(part 1 of 2)
# Autodesk Inventor assembly: NanoPower P31u-9
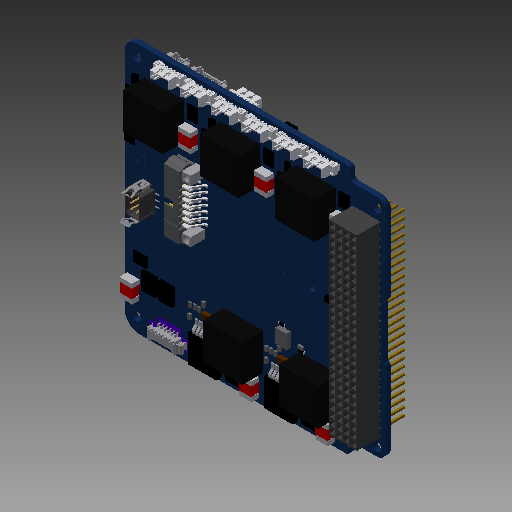
[picture p0: Inventor's stored thumbnail of the model, 512x512]
Saved by Autodesk Inventor 2017 (Build 210142000, 142)
## iProperties
Created: 2014-06-10
Part Number: NanoPower P31u-9
Document SubType Name: Assembly
Designer: Cosmonauta
Sending System: Autodesk Inventor 2014
Preprocessor: ST-DEVELOPER v15.2
Title: \\psf\Home\Desktop\NanoPower P31u-9.stp
Author: David
## Documents named in this file (322)
- C:\Users\Cosmonauta\ownCloud\Aurora\Proyectos\SUCHAI_2-3\Subsistemas\MEC\CAD_Cubesat3U\Nanopower_P31U\CAD\NanoPower P31u-9.iam
- C:\Users\Cosmonauta\ownCloud\Aurora\Proyectos\SUCHAI_2-3\Subsistemas\MEC\CAD_Cubesat3U\Nanopower_P31U\CAD\Board.ipt
- C:\Users\Cosmonauta\ownCloud\Aurora\Proyectos\SUCHAI_2-3\Subsistemas\MEC\CAD_Cubesat3U\Nanopower_P31U\CAD\R104.iam
- C:\Users\Cosmonauta\ownCloud\Aurora\Proyectos\SUCHAI_2-3\Subsistemas\MEC\CAD_Cubesat3U\Nanopower_P31U\CAD\R701.iam
- C:\Users\Cosmonauta\ownCloud\Aurora\Proyectos\SUCHAI_2-3\Subsistemas\MEC\CAD_Cubesat3U\Nanopower_P31U\CAD\U700.iam
- C:\Users\Cosmonauta\ownCloud\Aurora\Proyectos\SUCHAI_2-3\Subsistemas\MEC\CAD_Cubesat3U\Nanopower_P31U\CAD\R700.iam
- C:\Users\Cosmonauta\ownCloud\Aurora\Proyectos\SUCHAI_2-3\Subsistemas\MEC\CAD_Cubesat3U\Nanopower_P31U\CAD\C700.iam
- C:\Users\Cosmonauta\ownCloud\Aurora\Proyectos\SUCHAI_2-3\Subsistemas\MEC\CAD_Cubesat3U\Nanopower_P31U\CAD\Q411.iam
- C:\Users\Cosmonauta\ownCloud\Aurora\Proyectos\SUCHAI_2-3\Subsistemas\MEC\CAD_Cubesat3U\Nanopower_P31U\CAD\Q410.iam
- C:\Users\Cosmonauta\ownCloud\Aurora\Proyectos\SUCHAI_2-3\Subsistemas\MEC\CAD_Cubesat3U\Nanopower_P31U\CAD\U605.iam
- C:\Users\Cosmonauta\ownCloud\Aurora\Proyectos\SUCHAI_2-3\Subsistemas\MEC\CAD_Cubesat3U\Nanopower_P31U\CAD\U604.iam
- C:\Users\Cosmonauta\ownCloud\Aurora\Proyectos\SUCHAI_2-3\Subsistemas\MEC\CAD_Cubesat3U\Nanopower_P31U\CAD\U603.iam
- C:\Users\Cosmonauta\ownCloud\Aurora\Proyectos\SUCHAI_2-3\Subsistemas\MEC\CAD_Cubesat3U\Nanopower_P31U\CAD\U602.iam
- C:\Users\Cosmonauta\ownCloud\Aurora\Proyectos\SUCHAI_2-3\Subsistemas\MEC\CAD_Cubesat3U\Nanopower_P31U\CAD\R304.iam
- C:\Users\Cosmonauta\ownCloud\Aurora\Proyectos\SUCHAI_2-3\Subsistemas\MEC\CAD_Cubesat3U\Nanopower_P31U\CAD\R303.iam
- C:\Users\Cosmonauta\ownCloud\Aurora\Proyectos\SUCHAI_2-3\Subsistemas\MEC\CAD_Cubesat3U\Nanopower_P31U\CAD\R7_M506.iam
- C:\Users\Cosmonauta\ownCloud\Aurora\Proyectos\SUCHAI_2-3\Subsistemas\MEC\CAD_Cubesat3U\Nanopower_P31U\CAD\R7_M505.iam
- C:\Users\Cosmonauta\ownCloud\Aurora\Proyectos\SUCHAI_2-3\Subsistemas\MEC\CAD_Cubesat3U\Nanopower_P31U\CAD\R7_M504.iam
- C:\Users\Cosmonauta\ownCloud\Aurora\Proyectos\SUCHAI_2-3\Subsistemas\MEC\CAD_Cubesat3U\Nanopower_P31U\CAD\R7_M503.iam
- C:\Users\Cosmonauta\ownCloud\Aurora\Proyectos\SUCHAI_2-3\Subsistemas\MEC\CAD_Cubesat3U\Nanopower_P31U\CAD\R7_M502.iam
- C:\Users\Cosmonauta\ownCloud\Aurora\Proyectos\SUCHAI_2-3\Subsistemas\MEC\CAD_Cubesat3U\Nanopower_P31U\CAD\R7_M501.iam
- C:\Users\Cosmonauta\ownCloud\Aurora\Proyectos\SUCHAI_2-3\Subsistemas\MEC\CAD_Cubesat3U\Nanopower_P31U\CAD\C4_M506.iam
- C:\Users\Cosmonauta\ownCloud\Aurora\Proyectos\SUCHAI_2-3\Subsistemas\MEC\CAD_Cubesat3U\Nanopower_P31U\CAD\C4_M505.iam
- C:\Users\Cosmonauta\ownCloud\Aurora\Proyectos\SUCHAI_2-3\Subsistemas\MEC\CAD_Cubesat3U\Nanopower_P31U\CAD\C4_M504.iam
- C:\Users\Cosmonauta\ownCloud\Aurora\Proyectos\SUCHAI_2-3\Subsistemas\MEC\CAD_Cubesat3U\Nanopower_P31U\CAD\C4_M503.iam
- C:\Users\Cosmonauta\ownCloud\Aurora\Proyectos\SUCHAI_2-3\Subsistemas\MEC\CAD_Cubesat3U\Nanopower_P31U\CAD\C4_M502.iam
- C:\Users\Cosmonauta\ownCloud\Aurora\Proyectos\SUCHAI_2-3\Subsistemas\MEC\CAD_Cubesat3U\Nanopower_P31U\CAD\C4_M501.iam
- C:\Users\Cosmonauta\ownCloud\Aurora\Proyectos\SUCHAI_2-3\Subsistemas\MEC\CAD_Cubesat3U\Nanopower_P31U\CAD\R6_B3.iam
- C:\Users\Cosmonauta\ownCloud\Aurora\Proyectos\SUCHAI_2-3\Subsistemas\MEC\CAD_Cubesat3U\Nanopower_P31U\CAD\R6_B2.iam
- C:\Users\Cosmonauta\ownCloud\Aurora\Proyectos\SUCHAI_2-3\Subsistemas\MEC\CAD_Cubesat3U\Nanopower_P31U\CAD\R6_B1.iam
- C:\Users\Cosmonauta\ownCloud\Aurora\Proyectos\SUCHAI_2-3\Subsistemas\MEC\CAD_Cubesat3U\Nanopower_P31U\CAD\C6_B3.iam
- C:\Users\Cosmonauta\ownCloud\Aurora\Proyectos\SUCHAI_2-3\Subsistemas\MEC\CAD_Cubesat3U\Nanopower_P31U\CAD\C6_B2.iam
- C:\Users\Cosmonauta\ownCloud\Aurora\Proyectos\SUCHAI_2-3\Subsistemas\MEC\CAD_Cubesat3U\Nanopower_P31U\CAD\C6_B1.iam
- C:\Users\Cosmonauta\ownCloud\Aurora\Proyectos\SUCHAI_2-3\Subsistemas\MEC\CAD_Cubesat3U\Nanopower_P31U\CAD\R103.iam
- C:\Users\Cosmonauta\ownCloud\Aurora\Proyectos\SUCHAI_2-3\Subsistemas\MEC\CAD_Cubesat3U\Nanopower_P31U\CAD\R102.iam
- C:\Users\Cosmonauta\ownCloud\Aurora\Proyectos\SUCHAI_2-3\Subsistemas\MEC\CAD_Cubesat3U\Nanopower_P31U\CAD\C103.iam
- C:\Users\Cosmonauta\ownCloud\Aurora\Proyectos\SUCHAI_2-3\Subsistemas\MEC\CAD_Cubesat3U\Nanopower_P31U\CAD\C102.iam
- C:\Users\Cosmonauta\ownCloud\Aurora\Proyectos\SUCHAI_2-3\Subsistemas\MEC\CAD_Cubesat3U\Nanopower_P31U\CAD\R622.iam
- C:\Users\Cosmonauta\ownCloud\Aurora\Proyectos\SUCHAI_2-3\Subsistemas\MEC\CAD_Cubesat3U\Nanopower_P31U\CAD\R621.iam
- C:\Users\Cosmonauta\ownCloud\Aurora\Proyectos\SUCHAI_2-3\Subsistemas\MEC\CAD_Cubesat3U\Nanopower_P31U\CAD\R620.iam
- C:\Users\Cosmonauta\ownCloud\Aurora\Proyectos\SUCHAI_2-3\Subsistemas\MEC\CAD_Cubesat3U\Nanopower_P31U\CAD\R619.iam
- C:\Users\Cosmonauta\ownCloud\Aurora\Proyectos\SUCHAI_2-3\Subsistemas\MEC\CAD_Cubesat3U\Nanopower_P31U\CAD\R414.iam
- C:\Users\Cosmonauta\ownCloud\Aurora\Proyectos\SUCHAI_2-3\Subsistemas\MEC\CAD_Cubesat3U\Nanopower_P31U\CAD\P601.iam
- C:\Users\Cosmonauta\ownCloud\Aurora\Proyectos\SUCHAI_2-3\Subsistemas\MEC\CAD_Cubesat3U\Nanopower_P31U\CAD\U601.iam
- C:\Users\Cosmonauta\ownCloud\Aurora\Proyectos\SUCHAI_2-3\Subsistemas\MEC\CAD_Cubesat3U\Nanopower_P31U\CAD\P600.iam
- C:\Users\Cosmonauta\ownCloud\Aurora\Proyectos\SUCHAI_2-3\Subsistemas\MEC\CAD_Cubesat3U\Nanopower_P31U\CAD\PBAT.iam
- C:\Users\Cosmonauta\ownCloud\Aurora\Proyectos\SUCHAI_2-3\Subsistemas\MEC\CAD_Cubesat3U\Nanopower_P31U\CAD\C4_B50.iam
- C:\Users\Cosmonauta\ownCloud\Aurora\Proyectos\SUCHAI_2-3\Subsistemas\MEC\CAD_Cubesat3U\Nanopower_P31U\CAD\C2_B50.iam
- C:\Users\Cosmonauta\ownCloud\Aurora\Proyectos\SUCHAI_2-3\Subsistemas\MEC\CAD_Cubesat3U\Nanopower_P31U\CAD\U1_M506.iam
- C:\Users\Cosmonauta\ownCloud\Aurora\Proyectos\SUCHAI_2-3\Subsistemas\MEC\CAD_Cubesat3U\Nanopower_P31U\CAD\U1_M505.iam
- C:\Users\Cosmonauta\ownCloud\Aurora\Proyectos\SUCHAI_2-3\Subsistemas\MEC\CAD_Cubesat3U\Nanopower_P31U\CAD\U1_M504.iam
- C:\Users\Cosmonauta\ownCloud\Aurora\Proyectos\SUCHAI_2-3\Subsistemas\MEC\CAD_Cubesat3U\Nanopower_P31U\CAD\U1_M503.iam
- C:\Users\Cosmonauta\ownCloud\Aurora\Proyectos\SUCHAI_2-3\Subsistemas\MEC\CAD_Cubesat3U\Nanopower_P31U\CAD\U1_M502.iam
- C:\Users\Cosmonauta\ownCloud\Aurora\Proyectos\SUCHAI_2-3\Subsistemas\MEC\CAD_Cubesat3U\Nanopower_P31U\CAD\U1_M501.iam
- C:\Users\Cosmonauta\ownCloud\Aurora\Proyectos\SUCHAI_2-3\Subsistemas\MEC\CAD_Cubesat3U\Nanopower_P31U\CAD\C1_B1.iam
- C:\Users\Cosmonauta\ownCloud\Aurora\Proyectos\SUCHAI_2-3\Subsistemas\MEC\CAD_Cubesat3U\Nanopower_P31U\CAD\C1_B2.iam
- C:\Users\Cosmonauta\ownCloud\Aurora\Proyectos\SUCHAI_2-3\Subsistemas\MEC\CAD_Cubesat3U\Nanopower_P31U\CAD\C1_B3.iam
- C:\Users\Cosmonauta\ownCloud\Aurora\Proyectos\SUCHAI_2-3\Subsistemas\MEC\CAD_Cubesat3U\Nanopower_P31U\CAD\C2_B1.iam
- C:\Users\Cosmonauta\ownCloud\Aurora\Proyectos\SUCHAI_2-3\Subsistemas\MEC\CAD_Cubesat3U\Nanopower_P31U\CAD\C2_B2.iam
- C:\Users\Cosmonauta\ownCloud\Aurora\Proyectos\SUCHAI_2-3\Subsistemas\MEC\CAD_Cubesat3U\Nanopower_P31U\CAD\C2_B3.iam
- C:\Users\Cosmonauta\ownCloud\Aurora\Proyectos\SUCHAI_2-3\Subsistemas\MEC\CAD_Cubesat3U\Nanopower_P31U\CAD\C2_B33.iam
- C:\Users\Cosmonauta\ownCloud\Aurora\Proyectos\SUCHAI_2-3\Subsistemas\MEC\CAD_Cubesat3U\Nanopower_P31U\CAD\C3_B1.iam
- C:\Users\Cosmonauta\ownCloud\Aurora\Proyectos\SUCHAI_2-3\Subsistemas\MEC\CAD_Cubesat3U\Nanopower_P31U\CAD\C3_B2.iam
- C:\Users\Cosmonauta\ownCloud\Aurora\Proyectos\SUCHAI_2-3\Subsistemas\MEC\CAD_Cubesat3U\Nanopower_P31U\CAD\C3_B3.iam
- C:\Users\Cosmonauta\ownCloud\Aurora\Proyectos\SUCHAI_2-3\Subsistemas\MEC\CAD_Cubesat3U\Nanopower_P31U\CAD\C3_B33.iam
- C:\Users\Cosmonauta\ownCloud\Aurora\Proyectos\SUCHAI_2-3\Subsistemas\MEC\CAD_Cubesat3U\Nanopower_P31U\CAD\C3_B50.iam
- C:\Users\Cosmonauta\ownCloud\Aurora\Proyectos\SUCHAI_2-3\Subsistemas\MEC\CAD_Cubesat3U\Nanopower_P31U\CAD\C4_B1.iam
- C:\Users\Cosmonauta\ownCloud\Aurora\Proyectos\SUCHAI_2-3\Subsistemas\MEC\CAD_Cubesat3U\Nanopower_P31U\CAD\C4_B2.iam
- C:\Users\Cosmonauta\ownCloud\Aurora\Proyectos\SUCHAI_2-3\Subsistemas\MEC\CAD_Cubesat3U\Nanopower_P31U\CAD\C4_B3.iam
- C:\Users\Cosmonauta\ownCloud\Aurora\Proyectos\SUCHAI_2-3\Subsistemas\MEC\CAD_Cubesat3U\Nanopower_P31U\CAD\C4_B33.iam
- C:\Users\Cosmonauta\ownCloud\Aurora\Proyectos\SUCHAI_2-3\Subsistemas\MEC\CAD_Cubesat3U\Nanopower_P31U\CAD\C5_B33.iam
- C:\Users\Cosmonauta\ownCloud\Aurora\Proyectos\SUCHAI_2-3\Subsistemas\MEC\CAD_Cubesat3U\Nanopower_P31U\CAD\C5_B50.iam
- C:\Users\Cosmonauta\ownCloud\Aurora\Proyectos\SUCHAI_2-3\Subsistemas\MEC\CAD_Cubesat3U\Nanopower_P31U\CAD\C100.iam
- C:\Users\Cosmonauta\ownCloud\Aurora\Proyectos\SUCHAI_2-3\Subsistemas\MEC\CAD_Cubesat3U\Nanopower_P31U\CAD\C101.iam
- C:\Users\Cosmonauta\ownCloud\Aurora\Proyectos\SUCHAI_2-3\Subsistemas\MEC\CAD_Cubesat3U\Nanopower_P31U\CAD\C200.iam
- C:\Users\Cosmonauta\ownCloud\Aurora\Proyectos\SUCHAI_2-3\Subsistemas\MEC\CAD_Cubesat3U\Nanopower_P31U\CAD\C201.iam
- C:\Users\Cosmonauta\ownCloud\Aurora\Proyectos\SUCHAI_2-3\Subsistemas\MEC\CAD_Cubesat3U\Nanopower_P31U\CAD\C202.iam
- C:\Users\Cosmonauta\ownCloud\Aurora\Proyectos\SUCHAI_2-3\Subsistemas\MEC\CAD_Cubesat3U\Nanopower_P31U\CAD\C400.iam
- C:\Users\Cosmonauta\ownCloud\Aurora\Proyectos\SUCHAI_2-3\Subsistemas\MEC\CAD_Cubesat3U\Nanopower_P31U\CAD\D1_B1.iam
- C:\Users\Cosmonauta\ownCloud\Aurora\Proyectos\SUCHAI_2-3\Subsistemas\MEC\CAD_Cubesat3U\Nanopower_P31U\CAD\D1_B2.iam
- C:\Users\Cosmonauta\ownCloud\Aurora\Proyectos\SUCHAI_2-3\Subsistemas\MEC\CAD_Cubesat3U\Nanopower_P31U\CAD\D1_B3.iam
- C:\Users\Cosmonauta\ownCloud\Aurora\Proyectos\SUCHAI_2-3\Subsistemas\MEC\CAD_Cubesat3U\Nanopower_P31U\CAD\D1_B33.iam
- C:\Users\Cosmonauta\ownCloud\Aurora\Proyectos\SUCHAI_2-3\Subsistemas\MEC\CAD_Cubesat3U\Nanopower_P31U\CAD\D1_B50.iam
- C:\Users\Cosmonauta\ownCloud\Aurora\Proyectos\SUCHAI_2-3\Subsistemas\MEC\CAD_Cubesat3U\Nanopower_P31U\CAD\L1_B1.iam
- C:\Users\Cosmonauta\ownCloud\Aurora\Proyectos\SUCHAI_2-3\Subsistemas\MEC\CAD_Cubesat3U\Nanopower_P31U\CAD\L1_B2.iam
- C:\Users\Cosmonauta\ownCloud\Aurora\Proyectos\SUCHAI_2-3\Subsistemas\MEC\CAD_Cubesat3U\Nanopower_P31U\CAD\L1_B3.iam
- C:\Users\Cosmonauta\ownCloud\Aurora\Proyectos\SUCHAI_2-3\Subsistemas\MEC\CAD_Cubesat3U\Nanopower_P31U\CAD\L1_B33.iam
- C:\Users\Cosmonauta\ownCloud\Aurora\Proyectos\SUCHAI_2-3\Subsistemas\MEC\CAD_Cubesat3U\Nanopower_P31U\CAD\L1_B50.iam
- C:\Users\Cosmonauta\ownCloud\Aurora\Proyectos\SUCHAI_2-3\Subsistemas\MEC\CAD_Cubesat3U\Nanopower_P31U\CAD\P100.iam
- C:\Users\Cosmonauta\ownCloud\Aurora\Proyectos\SUCHAI_2-3\Subsistemas\MEC\CAD_Cubesat3U\Nanopower_P31U\CAD\P101.iam
- C:\Users\Cosmonauta\ownCloud\Aurora\Proyectos\SUCHAI_2-3\Subsistemas\MEC\CAD_Cubesat3U\Nanopower_P31U\CAD\P102.iam
- C:\Users\Cosmonauta\ownCloud\Aurora\Proyectos\SUCHAI_2-3\Subsistemas\MEC\CAD_Cubesat3U\Nanopower_P31U\CAD\P103.iam
- C:\Users\Cosmonauta\ownCloud\Aurora\Proyectos\SUCHAI_2-3\Subsistemas\MEC\CAD_Cubesat3U\Nanopower_P31U\CAD\P104.iam
- C:\Users\Cosmonauta\ownCloud\Aurora\Proyectos\SUCHAI_2-3\Subsistemas\MEC\CAD_Cubesat3U\Nanopower_P31U\CAD\P105.iam
- C:\Users\Cosmonauta\ownCloud\Aurora\Proyectos\SUCHAI_2-3\Subsistemas\MEC\CAD_Cubesat3U\Nanopower_P31U\CAD\P400.iam
- C:\Users\Cosmonauta\ownCloud\Aurora\Proyectos\SUCHAI_2-3\Subsistemas\MEC\CAD_Cubesat3U\Nanopower_P31U\CAD\Q1_B1.iam
- C:\Users\Cosmonauta\ownCloud\Aurora\Proyectos\SUCHAI_2-3\Subsistemas\MEC\CAD_Cubesat3U\Nanopower_P31U\CAD\Q1_B2.iam
- C:\Users\Cosmonauta\ownCloud\Aurora\Proyectos\SUCHAI_2-3\Subsistemas\MEC\CAD_Cubesat3U\Nanopower_P31U\CAD\Q1_B3.iam
- C:\Users\Cosmonauta\ownCloud\Aurora\Proyectos\SUCHAI_2-3\Subsistemas\MEC\CAD_Cubesat3U\Nanopower_P31U\CAD\Q2_B1.iam
- C:\Users\Cosmonauta\ownCloud\Aurora\Proyectos\SUCHAI_2-3\Subsistemas\MEC\CAD_Cubesat3U\Nanopower_P31U\CAD\Q2_B2.iam
- C:\Users\Cosmonauta\ownCloud\Aurora\Proyectos\SUCHAI_2-3\Subsistemas\MEC\CAD_Cubesat3U\Nanopower_P31U\CAD\Q2_B3.iam
- C:\Users\Cosmonauta\ownCloud\Aurora\Proyectos\SUCHAI_2-3\Subsistemas\MEC\CAD_Cubesat3U\Nanopower_P31U\CAD\Q200.iam
- C:\Users\Cosmonauta\ownCloud\Aurora\Proyectos\SUCHAI_2-3\Subsistemas\MEC\CAD_Cubesat3U\Nanopower_P31U\CAD\Q201.iam
- C:\Users\Cosmonauta\ownCloud\Aurora\Proyectos\SUCHAI_2-3\Subsistemas\MEC\CAD_Cubesat3U\Nanopower_P31U\CAD\Q400.iam
- C:\Users\Cosmonauta\ownCloud\Aurora\Proyectos\SUCHAI_2-3\Subsistemas\MEC\CAD_Cubesat3U\Nanopower_P31U\CAD\Q401.iam
- C:\Users\Cosmonauta\ownCloud\Aurora\Proyectos\SUCHAI_2-3\Subsistemas\MEC\CAD_Cubesat3U\Nanopower_P31U\CAD\Q402.iam
- C:\Users\Cosmonauta\ownCloud\Aurora\Proyectos\SUCHAI_2-3\Subsistemas\MEC\CAD_Cubesat3U\Nanopower_P31U\CAD\Q404.iam
- C:\Users\Cosmonauta\ownCloud\Aurora\Proyectos\SUCHAI_2-3\Subsistemas\MEC\CAD_Cubesat3U\Nanopower_P31U\CAD\R1_B1.iam
- C:\Users\Cosmonauta\ownCloud\Aurora\Proyectos\SUCHAI_2-3\Subsistemas\MEC\CAD_Cubesat3U\Nanopower_P31U\CAD\R1_B2.iam
- C:\Users\Cosmonauta\ownCloud\Aurora\Proyectos\SUCHAI_2-3\Subsistemas\MEC\CAD_Cubesat3U\Nanopower_P31U\CAD\R1_B3.iam
- C:\Users\Cosmonauta\ownCloud\Aurora\Proyectos\SUCHAI_2-3\Subsistemas\MEC\CAD_Cubesat3U\Nanopower_P31U\CAD\R1_B33.iam
- C:\Users\Cosmonauta\ownCloud\Aurora\Proyectos\SUCHAI_2-3\Subsistemas\MEC\CAD_Cubesat3U\Nanopower_P31U\CAD\R1_B50.iam
- C:\Users\Cosmonauta\ownCloud\Aurora\Proyectos\SUCHAI_2-3\Subsistemas\MEC\CAD_Cubesat3U\Nanopower_P31U\CAD\R2_B1.iam
- C:\Users\Cosmonauta\ownCloud\Aurora\Proyectos\SUCHAI_2-3\Subsistemas\MEC\CAD_Cubesat3U\Nanopower_P31U\CAD\R2_B2.iam
- C:\Users\Cosmonauta\ownCloud\Aurora\Proyectos\SUCHAI_2-3\Subsistemas\MEC\CAD_Cubesat3U\Nanopower_P31U\CAD\R2_B3.iam
- C:\Users\Cosmonauta\ownCloud\Aurora\Proyectos\SUCHAI_2-3\Subsistemas\MEC\CAD_Cubesat3U\Nanopower_P31U\CAD\R2_B33.iam
- C:\Users\Cosmonauta\ownCloud\Aurora\Proyectos\SUCHAI_2-3\Subsistemas\MEC\CAD_Cubesat3U\Nanopower_P31U\CAD\R2_B50.iam
- C:\Users\Cosmonauta\ownCloud\Aurora\Proyectos\SUCHAI_2-3\Subsistemas\MEC\CAD_Cubesat3U\Nanopower_P31U\CAD\R3_B1.iam
- C:\Users\Cosmonauta\ownCloud\Aurora\Proyectos\SUCHAI_2-3\Subsistemas\MEC\CAD_Cubesat3U\Nanopower_P31U\CAD\R3_B2.iam
- C:\Users\Cosmonauta\ownCloud\Aurora\Proyectos\SUCHAI_2-3\Subsistemas\MEC\CAD_Cubesat3U\Nanopower_P31U\CAD\R3_B3.iam
- C:\Users\Cosmonauta\ownCloud\Aurora\Proyectos\SUCHAI_2-3\Subsistemas\MEC\CAD_Cubesat3U\Nanopower_P31U\CAD\R3_B33.iam
- C:\Users\Cosmonauta\ownCloud\Aurora\Proyectos\SUCHAI_2-3\Subsistemas\MEC\CAD_Cubesat3U\Nanopower_P31U\CAD\R3_B50.iam
- C:\Users\Cosmonauta\ownCloud\Aurora\Proyectos\SUCHAI_2-3\Subsistemas\MEC\CAD_Cubesat3U\Nanopower_P31U\CAD\R4_B1.iam
- C:\Users\Cosmonauta\ownCloud\Aurora\Proyectos\SUCHAI_2-3\Subsistemas\MEC\CAD_Cubesat3U\Nanopower_P31U\CAD\R4_B2.iam
- C:\Users\Cosmonauta\ownCloud\Aurora\Proyectos\SUCHAI_2-3\Subsistemas\MEC\CAD_Cubesat3U\Nanopower_P31U\CAD\R4_B3.iam
- C:\Users\Cosmonauta\ownCloud\Aurora\Proyectos\SUCHAI_2-3\Subsistemas\MEC\CAD_Cubesat3U\Nanopower_P31U\CAD\R5_B1.iam
- C:\Users\Cosmonauta\ownCloud\Aurora\Proyectos\SUCHAI_2-3\Subsistemas\MEC\CAD_Cubesat3U\Nanopower_P31U\CAD\R5_B2.iam
- C:\Users\Cosmonauta\ownCloud\Aurora\Proyectos\SUCHAI_2-3\Subsistemas\MEC\CAD_Cubesat3U\Nanopower_P31U\CAD\R5_B3.iam
- C:\Users\Cosmonauta\ownCloud\Aurora\Proyectos\SUCHAI_2-3\Subsistemas\MEC\CAD_Cubesat3U\Nanopower_P31U\CAD\R100.iam
- C:\Users\Cosmonauta\ownCloud\Aurora\Proyectos\SUCHAI_2-3\Subsistemas\MEC\CAD_Cubesat3U\Nanopower_P31U\CAD\R101.iam
- C:\Users\Cosmonauta\ownCloud\Aurora\Proyectos\SUCHAI_2-3\Subsistemas\MEC\CAD_Cubesat3U\Nanopower_P31U\CAD\R107_B1.iam
- C:\Users\Cosmonauta\ownCloud\Aurora\Proyectos\SUCHAI_2-3\Subsistemas\MEC\CAD_Cubesat3U\Nanopower_P31U\CAD\R107_B2.iam
- C:\Users\Cosmonauta\ownCloud\Aurora\Proyectos\SUCHAI_2-3\Subsistemas\MEC\CAD_Cubesat3U\Nanopower_P31U\CAD\R107_B3.iam
- C:\Users\Cosmonauta\ownCloud\Aurora\Proyectos\SUCHAI_2-3\Subsistemas\MEC\CAD_Cubesat3U\Nanopower_P31U\CAD\R200.iam
- C:\Users\Cosmonauta\ownCloud\Aurora\Proyectos\SUCHAI_2-3\Subsistemas\MEC\CAD_Cubesat3U\Nanopower_P31U\CAD\R201.iam
- C:\Users\Cosmonauta\ownCloud\Aurora\Proyectos\SUCHAI_2-3\Subsistemas\MEC\CAD_Cubesat3U\Nanopower_P31U\CAD\R202.iam
- C:\Users\Cosmonauta\ownCloud\Aurora\Proyectos\SUCHAI_2-3\Subsistemas\MEC\CAD_Cubesat3U\Nanopower_P31U\CAD\R203.iam
- C:\Users\Cosmonauta\ownCloud\Aurora\Proyectos\SUCHAI_2-3\Subsistemas\MEC\CAD_Cubesat3U\Nanopower_P31U\CAD\R204.iam
- C:\Users\Cosmonauta\ownCloud\Aurora\Proyectos\SUCHAI_2-3\Subsistemas\MEC\CAD_Cubesat3U\Nanopower_P31U\CAD\R205.iam
- C:\Users\Cosmonauta\ownCloud\Aurora\Proyectos\SUCHAI_2-3\Subsistemas\MEC\CAD_Cubesat3U\Nanopower_P31U\CAD\R206.iam
- C:\Users\Cosmonauta\ownCloud\Aurora\Proyectos\SUCHAI_2-3\Subsistemas\MEC\CAD_Cubesat3U\Nanopower_P31U\CAD\R207.iam
- C:\Users\Cosmonauta\ownCloud\Aurora\Proyectos\SUCHAI_2-3\Subsistemas\MEC\CAD_Cubesat3U\Nanopower_P31U\CAD\R208.iam
- C:\Users\Cosmonauta\ownCloud\Aurora\Proyectos\SUCHAI_2-3\Subsistemas\MEC\CAD_Cubesat3U\Nanopower_P31U\CAD\R209.iam
- C:\Users\Cosmonauta\ownCloud\Aurora\Proyectos\SUCHAI_2-3\Subsistemas\MEC\CAD_Cubesat3U\Nanopower_P31U\CAD\R210.iam
- C:\Users\Cosmonauta\ownCloud\Aurora\Proyectos\SUCHAI_2-3\Subsistemas\MEC\CAD_Cubesat3U\Nanopower_P31U\CAD\R400.iam
- C:\Users\Cosmonauta\ownCloud\Aurora\Proyectos\SUCHAI_2-3\Subsistemas\MEC\CAD_Cubesat3U\Nanopower_P31U\CAD\R401.iam
- C:\Users\Cosmonauta\ownCloud\Aurora\Proyectos\SUCHAI_2-3\Subsistemas\MEC\CAD_Cubesat3U\Nanopower_P31U\CAD\R402.iam
- C:\Users\Cosmonauta\ownCloud\Aurora\Proyectos\SUCHAI_2-3\Subsistemas\MEC\CAD_Cubesat3U\Nanopower_P31U\CAD\R403.iam
- C:\Users\Cosmonauta\ownCloud\Aurora\Proyectos\SUCHAI_2-3\Subsistemas\MEC\CAD_Cubesat3U\Nanopower_P31U\CAD\R404.iam
- C:\Users\Cosmonauta\ownCloud\Aurora\Proyectos\SUCHAI_2-3\Subsistemas\MEC\CAD_Cubesat3U\Nanopower_P31U\CAD\R405.iam
- C:\Users\Cosmonauta\ownCloud\Aurora\Proyectos\SUCHAI_2-3\Subsistemas\MEC\CAD_Cubesat3U\Nanopower_P31U\CAD\R406.iam
- C:\Users\Cosmonauta\ownCloud\Aurora\Proyectos\SUCHAI_2-3\Subsistemas\MEC\CAD_Cubesat3U\Nanopower_P31U\CAD\R407.iam
- C:\Users\Cosmonauta\ownCloud\Aurora\Proyectos\SUCHAI_2-3\Subsistemas\MEC\CAD_Cubesat3U\Nanopower_P31U\CAD\R408.iam
- C:\Users\Cosmonauta\ownCloud\Aurora\Proyectos\SUCHAI_2-3\Subsistemas\MEC\CAD_Cubesat3U\Nanopower_P31U\CAD\R409.iam
- C:\Users\Cosmonauta\ownCloud\Aurora\Proyectos\SUCHAI_2-3\Subsistemas\MEC\CAD_Cubesat3U\Nanopower_P31U\CAD\R410.iam
- C:\Users\Cosmonauta\ownCloud\Aurora\Proyectos\SUCHAI_2-3\Subsistemas\MEC\CAD_Cubesat3U\Nanopower_P31U\CAD\R411.iam
- C:\Users\Cosmonauta\ownCloud\Aurora\Proyectos\SUCHAI_2-3\Subsistemas\MEC\CAD_Cubesat3U\Nanopower_P31U\CAD\U1_B1.iam
- C:\Users\Cosmonauta\ownCloud\Aurora\Proyectos\SUCHAI_2-3\Subsistemas\MEC\CAD_Cubesat3U\Nanopower_P31U\CAD\U1_B2.iam
- C:\Users\Cosmonauta\ownCloud\Aurora\Proyectos\SUCHAI_2-3\Subsistemas\MEC\CAD_Cubesat3U\Nanopower_P31U\CAD\U1_B3.iam
- C:\Users\Cosmonauta\ownCloud\Aurora\Proyectos\SUCHAI_2-3\Subsistemas\MEC\CAD_Cubesat3U\Nanopower_P31U\CAD\U1_B33.iam
- C:\Users\Cosmonauta\ownCloud\Aurora\Proyectos\SUCHAI_2-3\Subsistemas\MEC\CAD_Cubesat3U\Nanopower_P31U\CAD\U1_B50.iam
- C:\Users\Cosmonauta\ownCloud\Aurora\Proyectos\SUCHAI_2-3\Subsistemas\MEC\CAD_Cubesat3U\Nanopower_P31U\CAD\U2_B1.iam
- C:\Users\Cosmonauta\ownCloud\Aurora\Proyectos\SUCHAI_2-3\Subsistemas\MEC\CAD_Cubesat3U\Nanopower_P31U\CAD\U2_B2.iam
- C:\Users\Cosmonauta\ownCloud\Aurora\Proyectos\SUCHAI_2-3\Subsistemas\MEC\CAD_Cubesat3U\Nanopower_P31U\CAD\U2_B3.iam
- C:\Users\Cosmonauta\ownCloud\Aurora\Proyectos\SUCHAI_2-3\Subsistemas\MEC\CAD_Cubesat3U\Nanopower_P31U\CAD\U100.iam
- C:\Users\Cosmonauta\ownCloud\Aurora\Proyectos\SUCHAI_2-3\Subsistemas\MEC\CAD_Cubesat3U\Nanopower_P31U\CAD\U101.iam
- C:\Users\Cosmonauta\ownCloud\Aurora\Proyectos\SUCHAI_2-3\Subsistemas\MEC\CAD_Cubesat3U\Nanopower_P31U\CAD\U200.iam
- C:\Users\Cosmonauta\ownCloud\Aurora\Proyectos\SUCHAI_2-3\Subsistemas\MEC\CAD_Cubesat3U\Nanopower_P31U\CAD\U201.iam
- C:\Users\Cosmonauta\ownCloud\Aurora\Proyectos\SUCHAI_2-3\Subsistemas\MEC\CAD_Cubesat3U\Nanopower_P31U\CAD\C1_M501.iam
- C:\Users\Cosmonauta\ownCloud\Aurora\Proyectos\SUCHAI_2-3\Subsistemas\MEC\CAD_Cubesat3U\Nanopower_P31U\CAD\C1_M502.iam
- C:\Users\Cosmonauta\ownCloud\Aurora\Proyectos\SUCHAI_2-3\Subsistemas\MEC\CAD_Cubesat3U\Nanopower_P31U\CAD\C1_M503.iam
- C:\Users\Cosmonauta\ownCloud\Aurora\Proyectos\SUCHAI_2-3\Subsistemas\MEC\CAD_Cubesat3U\Nanopower_P31U\CAD\C1_M504.iam
- C:\Users\Cosmonauta\ownCloud\Aurora\Proyectos\SUCHAI_2-3\Subsistemas\MEC\CAD_Cubesat3U\Nanopower_P31U\CAD\C1_M505.iam
- C:\Users\Cosmonauta\ownCloud\Aurora\Proyectos\SUCHAI_2-3\Subsistemas\MEC\CAD_Cubesat3U\Nanopower_P31U\CAD\C1_M506.iam
- C:\Users\Cosmonauta\ownCloud\Aurora\Proyectos\SUCHAI_2-3\Subsistemas\MEC\CAD_Cubesat3U\Nanopower_P31U\CAD\C2_M501.iam
- C:\Users\Cosmonauta\ownCloud\Aurora\Proyectos\SUCHAI_2-3\Subsistemas\MEC\CAD_Cubesat3U\Nanopower_P31U\CAD\C2_M502.iam
- C:\Users\Cosmonauta\ownCloud\Aurora\Proyectos\SUCHAI_2-3\Subsistemas\MEC\CAD_Cubesat3U\Nanopower_P31U\CAD\C2_M503.iam
- C:\Users\Cosmonauta\ownCloud\Aurora\Proyectos\SUCHAI_2-3\Subsistemas\MEC\CAD_Cubesat3U\Nanopower_P31U\CAD\C2_M504.iam
- C:\Users\Cosmonauta\ownCloud\Aurora\Proyectos\SUCHAI_2-3\Subsistemas\MEC\CAD_Cubesat3U\Nanopower_P31U\CAD\C2_M505.iam
- C:\Users\Cosmonauta\ownCloud\Aurora\Proyectos\SUCHAI_2-3\Subsistemas\MEC\CAD_Cubesat3U\Nanopower_P31U\CAD\C2_M506.iam
- C:\Users\Cosmonauta\ownCloud\Aurora\Proyectos\SUCHAI_2-3\Subsistemas\MEC\CAD_Cubesat3U\Nanopower_P31U\CAD\C3_M501.iam
- C:\Users\Cosmonauta\ownCloud\Aurora\Proyectos\SUCHAI_2-3\Subsistemas\MEC\CAD_Cubesat3U\Nanopower_P31U\CAD\C3_M502.iam
- C:\Users\Cosmonauta\ownCloud\Aurora\Proyectos\SUCHAI_2-3\Subsistemas\MEC\CAD_Cubesat3U\Nanopower_P31U\CAD\C3_M503.iam
- C:\Users\Cosmonauta\ownCloud\Aurora\Proyectos\SUCHAI_2-3\Subsistemas\MEC\CAD_Cubesat3U\Nanopower_P31U\CAD\C3_M504.iam
- C:\Users\Cosmonauta\ownCloud\Aurora\Proyectos\SUCHAI_2-3\Subsistemas\MEC\CAD_Cubesat3U\Nanopower_P31U\CAD\C3_M505.iam
- C:\Users\Cosmonauta\ownCloud\Aurora\Proyectos\SUCHAI_2-3\Subsistemas\MEC\CAD_Cubesat3U\Nanopower_P31U\CAD\C3_M506.iam
- C:\Users\Cosmonauta\ownCloud\Aurora\Proyectos\SUCHAI_2-3\Subsistemas\MEC\CAD_Cubesat3U\Nanopower_P31U\CAD\R1_M501.iam
- C:\Users\Cosmonauta\ownCloud\Aurora\Proyectos\SUCHAI_2-3\Subsistemas\MEC\CAD_Cubesat3U\Nanopower_P31U\CAD\R1_M502.iam
- C:\Users\Cosmonauta\ownCloud\Aurora\Proyectos\SUCHAI_2-3\Subsistemas\MEC\CAD_Cubesat3U\Nanopower_P31U\CAD\R1_M503.iam
- C:\Users\Cosmonauta\ownCloud\Aurora\Proyectos\SUCHAI_2-3\Subsistemas\MEC\CAD_Cubesat3U\Nanopower_P31U\CAD\R1_M504.iam
- C:\Users\Cosmonauta\ownCloud\Aurora\Proyectos\SUCHAI_2-3\Subsistemas\MEC\CAD_Cubesat3U\Nanopower_P31U\CAD\R1_M505.iam
- C:\Users\Cosmonauta\ownCloud\Aurora\Proyectos\SUCHAI_2-3\Subsistemas\MEC\CAD_Cubesat3U\Nanopower_P31U\CAD\R1_M506.iam
- C:\Users\Cosmonauta\ownCloud\Aurora\Proyectos\SUCHAI_2-3\Subsistemas\MEC\CAD_Cubesat3U\Nanopower_P31U\CAD\R2_M501.iam
- C:\Users\Cosmonauta\ownCloud\Aurora\Proyectos\SUCHAI_2-3\Subsistemas\MEC\CAD_Cubesat3U\Nanopower_P31U\CAD\R2_M502.iam
- C:\Users\Cosmonauta\ownCloud\Aurora\Proyectos\SUCHAI_2-3\Subsistemas\MEC\CAD_Cubesat3U\Nanopower_P31U\CAD\R2_M503.iam
- C:\Users\Cosmonauta\ownCloud\Aurora\Proyectos\SUCHAI_2-3\Subsistemas\MEC\CAD_Cubesat3U\Nanopower_P31U\CAD\R2_M504.iam
- C:\Users\Cosmonauta\ownCloud\Aurora\Proyectos\SUCHAI_2-3\Subsistemas\MEC\CAD_Cubesat3U\Nanopower_P31U\CAD\R2_M505.iam
- C:\Users\Cosmonauta\ownCloud\Aurora\Proyectos\SUCHAI_2-3\Subsistemas\MEC\CAD_Cubesat3U\Nanopower_P31U\CAD\R2_M506.iam
- C:\Users\Cosmonauta\ownCloud\Aurora\Proyectos\SUCHAI_2-3\Subsistemas\MEC\CAD_Cubesat3U\Nanopower_P31U\CAD\R3_M501.iam
- C:\Users\Cosmonauta\ownCloud\Aurora\Proyectos\SUCHAI_2-3\Subsistemas\MEC\CAD_Cubesat3U\Nanopower_P31U\CAD\R3_M502.iam
- C:\Users\Cosmonauta\ownCloud\Aurora\Proyectos\SUCHAI_2-3\Subsistemas\MEC\CAD_Cubesat3U\Nanopower_P31U\CAD\R3_M503.iam
- C:\Users\Cosmonauta\ownCloud\Aurora\Proyectos\SUCHAI_2-3\Subsistemas\MEC\CAD_Cubesat3U\Nanopower_P31U\CAD\R3_M504.iam
- C:\Users\Cosmonauta\ownCloud\Aurora\Proyectos\SUCHAI_2-3\Subsistemas\MEC\CAD_Cubesat3U\Nanopower_P31U\CAD\R3_M505.iam
- C:\Users\Cosmonauta\ownCloud\Aurora\Proyectos\SUCHAI_2-3\Subsistemas\MEC\CAD_Cubesat3U\Nanopower_P31U\CAD\R3_M506.iam
- C:\Users\Cosmonauta\ownCloud\Aurora\Proyectos\SUCHAI_2-3\Subsistemas\MEC\CAD_Cubesat3U\Nanopower_P31U\CAD\R4_M501.iam
- C:\Users\Cosmonauta\ownCloud\Aurora\Proyectos\SUCHAI_2-3\Subsistemas\MEC\CAD_Cubesat3U\Nanopower_P31U\CAD\R4_M502.iam
- C:\Users\Cosmonauta\ownCloud\Aurora\Proyectos\SUCHAI_2-3\Subsistemas\MEC\CAD_Cubesat3U\Nanopower_P31U\CAD\R4_M503.iam
- C:\Users\Cosmonauta\ownCloud\Aurora\Proyectos\SUCHAI_2-3\Subsistemas\MEC\CAD_Cubesat3U\Nanopower_P31U\CAD\R4_M504.iam
- C:\Users\Cosmonauta\ownCloud\Aurora\Proyectos\SUCHAI_2-3\Subsistemas\MEC\CAD_Cubesat3U\Nanopower_P31U\CAD\R4_M505.iam
- C:\Users\Cosmonauta\ownCloud\Aurora\Proyectos\SUCHAI_2-3\Subsistemas\MEC\CAD_Cubesat3U\Nanopower_P31U\CAD\R4_M506.iam
- C:\Users\Cosmonauta\ownCloud\Aurora\Proyectos\SUCHAI_2-3\Subsistemas\MEC\CAD_Cubesat3U\Nanopower_P31U\CAD\R5_M501.iam
- C:\Users\Cosmonauta\ownCloud\Aurora\Proyectos\SUCHAI_2-3\Subsistemas\MEC\CAD_Cubesat3U\Nanopower_P31U\CAD\R5_M502.iam
- C:\Users\Cosmonauta\ownCloud\Aurora\Proyectos\SUCHAI_2-3\Subsistemas\MEC\CAD_Cubesat3U\Nanopower_P31U\CAD\R5_M503.iam
- C:\Users\Cosmonauta\ownCloud\Aurora\Proyectos\SUCHAI_2-3\Subsistemas\MEC\CAD_Cubesat3U\Nanopower_P31U\CAD\R5_M504.iam
- C:\Users\Cosmonauta\ownCloud\Aurora\Proyectos\SUCHAI_2-3\Subsistemas\MEC\CAD_Cubesat3U\Nanopower_P31U\CAD\R5_M505.iam
- C:\Users\Cosmonauta\ownCloud\Aurora\Proyectos\SUCHAI_2-3\Subsistemas\MEC\CAD_Cubesat3U\Nanopower_P31U\CAD\R5_M506.iam
- C:\Users\Cosmonauta\ownCloud\Aurora\Proyectos\SUCHAI_2-3\Subsistemas\MEC\CAD_Cubesat3U\Nanopower_P31U\CAD\R6_M501.iam
- C:\Users\Cosmonauta\ownCloud\Aurora\Proyectos\SUCHAI_2-3\Subsistemas\MEC\CAD_Cubesat3U\Nanopower_P31U\CAD\R6_M502.iam
- C:\Users\Cosmonauta\ownCloud\Aurora\Proyectos\SUCHAI_2-3\Subsistemas\MEC\CAD_Cubesat3U\Nanopower_P31U\CAD\R6_M503.iam
- C:\Users\Cosmonauta\ownCloud\Aurora\Proyectos\SUCHAI_2-3\Subsistemas\MEC\CAD_Cubesat3U\Nanopower_P31U\CAD\R6_M504.iam
- C:\Users\Cosmonauta\ownCloud\Aurora\Proyectos\SUCHAI_2-3\Subsistemas\MEC\CAD_Cubesat3U\Nanopower_P31U\CAD\R6_M505.iam
- C:\Users\Cosmonauta\ownCloud\Aurora\Proyectos\SUCHAI_2-3\Subsistemas\MEC\CAD_Cubesat3U\Nanopower_P31U\CAD\R6_M506.iam
- C:\Users\Cosmonauta\ownCloud\Aurora\Proyectos\SUCHAI_2-3\Subsistemas\MEC\CAD_Cubesat3U\Nanopower_P31U\CAD\U2_M501.iam
- C:\Users\Cosmonauta\ownCloud\Aurora\Proyectos\SUCHAI_2-3\Subsistemas\MEC\CAD_Cubesat3U\Nanopower_P31U\CAD\U2_M502.iam
- C:\Users\Cosmonauta\ownCloud\Aurora\Proyectos\SUCHAI_2-3\Subsistemas\MEC\CAD_Cubesat3U\Nanopower_P31U\CAD\U2_M503.iam
- C:\Users\Cosmonauta\ownCloud\Aurora\Proyectos\SUCHAI_2-3\Subsistemas\MEC\CAD_Cubesat3U\Nanopower_P31U\CAD\U2_M504.iam
- C:\Users\Cosmonauta\ownCloud\Aurora\Proyectos\SUCHAI_2-3\Subsistemas\MEC\CAD_Cubesat3U\Nanopower_P31U\CAD\U2_M505.iam
- C:\Users\Cosmonauta\ownCloud\Aurora\Proyectos\SUCHAI_2-3\Subsistemas\MEC\CAD_Cubesat3U\Nanopower_P31U\CAD\U2_M506.iam
- C:\Users\Cosmonauta\ownCloud\Aurora\Proyectos\SUCHAI_2-3\Subsistemas\MEC\CAD_Cubesat3U\Nanopower_P31U\CAD\C600.iam
- C:\Users\Cosmonauta\ownCloud\Aurora\Proyectos\SUCHAI_2-3\Subsistemas\MEC\CAD_Cubesat3U\Nanopower_P31U\CAD\R600.iam
- C:\Users\Cosmonauta\ownCloud\Aurora\Proyectos\SUCHAI_2-3\Subsistemas\MEC\CAD_Cubesat3U\Nanopower_P31U\CAD\U600.iam
- C:\Users\Cosmonauta\ownCloud\Aurora\Proyectos\SUCHAI_2-3\Subsistemas\MEC\CAD_Cubesat3U\Nanopower_P31U\CAD\C500.iam
- C:\Users\Cosmonauta\ownCloud\Aurora\Proyectos\SUCHAI_2-3\Subsistemas\MEC\CAD_Cubesat3U\Nanopower_P31U\CAD\C501.iam
- C:\Users\Cosmonauta\ownCloud\Aurora\Proyectos\SUCHAI_2-3\Subsistemas\MEC\CAD_Cubesat3U\Nanopower_P31U\CAD\C502.iam
- C:\Users\Cosmonauta\ownCloud\Aurora\Proyectos\SUCHAI_2-3\Subsistemas\MEC\CAD_Cubesat3U\Nanopower_P31U\CAD\C503.iam
- C:\Users\Cosmonauta\ownCloud\Aurora\Proyectos\SUCHAI_2-3\Subsistemas\MEC\CAD_Cubesat3U\Nanopower_P31U\CAD\C504.iam
- C:\Users\Cosmonauta\ownCloud\Aurora\Proyectos\SUCHAI_2-3\Subsistemas\MEC\CAD_Cubesat3U\Nanopower_P31U\CAD\C601.iam
- C:\Users\Cosmonauta\ownCloud\Aurora\Proyectos\SUCHAI_2-3\Subsistemas\MEC\CAD_Cubesat3U\Nanopower_P31U\CAD\C602.iam
- C:\Users\Cosmonauta\ownCloud\Aurora\Proyectos\SUCHAI_2-3\Subsistemas\MEC\CAD_Cubesat3U\Nanopower_P31U\CAD\C603.iam
- C:\Users\Cosmonauta\ownCloud\Aurora\Proyectos\SUCHAI_2-3\Subsistemas\MEC\CAD_Cubesat3U\Nanopower_P31U\CAD\C604.iam
- C:\Users\Cosmonauta\ownCloud\Aurora\Proyectos\SUCHAI_2-3\Subsistemas\MEC\CAD_Cubesat3U\Nanopower_P31U\CAD\R500.iam
- C:\Users\Cosmonauta\ownCloud\Aurora\Proyectos\SUCHAI_2-3\Subsistemas\MEC\CAD_Cubesat3U\Nanopower_P31U\CAD\R501.iam
- C:\Users\Cosmonauta\ownCloud\Aurora\Proyectos\SUCHAI_2-3\Subsistemas\MEC\CAD_Cubesat3U\Nanopower_P31U\CAD\R502.iam
- C:\Users\Cosmonauta\ownCloud\Aurora\Proyectos\SUCHAI_2-3\Subsistemas\MEC\CAD_Cubesat3U\Nanopower_P31U\CAD\R503.iam
- C:\Users\Cosmonauta\ownCloud\Aurora\Proyectos\SUCHAI_2-3\Subsistemas\MEC\CAD_Cubesat3U\Nanopower_P31U\CAD\R504.iam
- C:\Users\Cosmonauta\ownCloud\Aurora\Proyectos\SUCHAI_2-3\Subsistemas\MEC\CAD_Cubesat3U\Nanopower_P31U\CAD\R505.iam
- C:\Users\Cosmonauta\ownCloud\Aurora\Proyectos\SUCHAI_2-3\Subsistemas\MEC\CAD_Cubesat3U\Nanopower_P31U\CAD\R506.iam
- C:\Users\Cosmonauta\ownCloud\Aurora\Proyectos\SUCHAI_2-3\Subsistemas\MEC\CAD_Cubesat3U\Nanopower_P31U\CAD\R507.iam
- C:\Users\Cosmonauta\ownCloud\Aurora\Proyectos\SUCHAI_2-3\Subsistemas\MEC\CAD_Cubesat3U\Nanopower_P31U\CAD\U500.iam
- C:\Users\Cosmonauta\ownCloud\Aurora\Proyectos\SUCHAI_2-3\Subsistemas\MEC\CAD_Cubesat3U\Nanopower_P31U\CAD\TMP1.iam
- C:\Users\Cosmonauta\ownCloud\Aurora\Proyectos\SUCHAI_2-3\Subsistemas\MEC\CAD_Cubesat3U\Nanopower_P31U\CAD\TMP2.iam
- C:\Users\Cosmonauta\ownCloud\Aurora\Proyectos\SUCHAI_2-3\Subsistemas\MEC\CAD_Cubesat3U\Nanopower_P31U\CAD\TMP3.iam
- C:\Users\Cosmonauta\ownCloud\Aurora\Proyectos\SUCHAI_2-3\Subsistemas\MEC\CAD_Cubesat3U\Nanopower_P31U\CAD\TMP4.iam
- C:\Users\Cosmonauta\ownCloud\Aurora\Proyectos\SUCHAI_2-3\Subsistemas\MEC\CAD_Cubesat3U\Nanopower_P31U\CAD\C5_B1.iam
- C:\Users\Cosmonauta\ownCloud\Aurora\Proyectos\SUCHAI_2-3\Subsistemas\MEC\CAD_Cubesat3U\Nanopower_P31U\CAD\C5_B2.iam
- C:\Users\Cosmonauta\ownCloud\Aurora\Proyectos\SUCHAI_2-3\Subsistemas\MEC\CAD_Cubesat3U\Nanopower_P31U\CAD\C5_B3.iam
- C:\Users\Cosmonauta\ownCloud\Aurora\Proyectos\SUCHAI_2-3\Subsistemas\MEC\CAD_Cubesat3U\Nanopower_P31U\CAD\C203.iam
- C:\Users\Cosmonauta\ownCloud\Aurora\Proyectos\SUCHAI_2-3\Subsistemas\MEC\CAD_Cubesat3U\Nanopower_P31U\CAD\C204.iam
- C:\Users\Cosmonauta\ownCloud\Aurora\Proyectos\SUCHAI_2-3\Subsistemas\MEC\CAD_Cubesat3U\Nanopower_P31U\CAD\C800.iam
- C:\Users\Cosmonauta\ownCloud\Aurora\Proyectos\SUCHAI_2-3\Subsistemas\MEC\CAD_Cubesat3U\Nanopower_P31U\CAD\C801.iam
- C:\Users\Cosmonauta\ownCloud\Aurora\Proyectos\SUCHAI_2-3\Subsistemas\MEC\CAD_Cubesat3U\Nanopower_P31U\CAD\C802.iam
- C:\Users\Cosmonauta\ownCloud\Aurora\Proyectos\SUCHAI_2-3\Subsistemas\MEC\CAD_Cubesat3U\Nanopower_P31U\CAD\D802.iam
- C:\Users\Cosmonauta\ownCloud\Aurora\Proyectos\SUCHAI_2-3\Subsistemas\MEC\CAD_Cubesat3U\Nanopower_P31U\CAD\L800.iam
- C:\Users\Cosmonauta\ownCloud\Aurora\Proyectos\SUCHAI_2-3\Subsistemas\MEC\CAD_Cubesat3U\Nanopower_P31U\CAD\Q800.iam
- C:\Users\Cosmonauta\ownCloud\Aurora\Proyectos\SUCHAI_2-3\Subsistemas\MEC\CAD_Cubesat3U\Nanopower_P31U\CAD\Q801.iam
- C:\Users\Cosmonauta\ownCloud\Aurora\Proyectos\SUCHAI_2-3\Subsistemas\MEC\CAD_Cubesat3U\Nanopower_P31U\CAD\Q802.iam
- C:\Users\Cosmonauta\ownCloud\Aurora\Proyectos\SUCHAI_2-3\Subsistemas\MEC\CAD_Cubesat3U\Nanopower_P31U\CAD\R800.iam
- C:\Users\Cosmonauta\ownCloud\Aurora\Proyectos\SUCHAI_2-3\Subsistemas\MEC\CAD_Cubesat3U\Nanopower_P31U\CAD\R801.iam
- C:\Users\Cosmonauta\ownCloud\Aurora\Proyectos\SUCHAI_2-3\Subsistemas\MEC\CAD_Cubesat3U\Nanopower_P31U\CAD\R802.iam
- C:\Users\Cosmonauta\ownCloud\Aurora\Proyectos\SUCHAI_2-3\Subsistemas\MEC\CAD_Cubesat3U\Nanopower_P31U\CAD\R803.iam
- C:\Users\Cosmonauta\ownCloud\Aurora\Proyectos\SUCHAI_2-3\Subsistemas\MEC\CAD_Cubesat3U\Nanopower_P31U\CAD\R804.iam
- C:\Users\Cosmonauta\ownCloud\Aurora\Proyectos\SUCHAI_2-3\Subsistemas\MEC\CAD_Cubesat3U\Nanopower_P31U\CAD\U800.iam
- C:\Users\Cosmonauta\ownCloud\Aurora\Proyectos\SUCHAI_2-3\Subsistemas\MEC\CAD_Cubesat3U\Nanopower_P31U\CAD\C401.iam
- C:\Users\Cosmonauta\ownCloud\Aurora\Proyectos\SUCHAI_2-3\Subsistemas\MEC\CAD_Cubesat3U\Nanopower_P31U\CAD\Q406.iam
- C:\Users\Cosmonauta\ownCloud\Aurora\Proyectos\SUCHAI_2-3\Subsistemas\MEC\CAD_Cubesat3U\Nanopower_P31U\CAD\R413.iam
- C:\Users\Cosmonauta\ownCloud\Aurora\Proyectos\SUCHAI_2-3\Subsistemas\MEC\CAD_Cubesat3U\Nanopower_P31U\CAD\R601.iam
- C:\Users\Cosmonauta\ownCloud\Aurora\Proyectos\SUCHAI_2-3\Subsistemas\MEC\CAD_Cubesat3U\Nanopower_P31U\CAD\R602.iam
- C:\Users\Cosmonauta\ownCloud\Aurora\Proyectos\SUCHAI_2-3\Subsistemas\MEC\CAD_Cubesat3U\Nanopower_P31U\CAD\R603.iam
- C:\Users\Cosmonauta\ownCloud\Aurora\Proyectos\SUCHAI_2-3\Subsistemas\MEC\CAD_Cubesat3U\Nanopower_P31U\CAD\R604.iam
- C:\Users\Cosmonauta\ownCloud\Aurora\Proyectos\SUCHAI_2-3\Subsistemas\MEC\CAD_Cubesat3U\Nanopower_P31U\CAD\R605.iam
- C:\Users\Cosmonauta\ownCloud\Aurora\Proyectos\SUCHAI_2-3\Subsistemas\MEC\CAD_Cubesat3U\Nanopower_P31U\CAD\R606.iam
- C:\Users\Cosmonauta\ownCloud\Aurora\Proyectos\SUCHAI_2-3\Subsistemas\MEC\CAD_Cubesat3U\Nanopower_P31U\CAD\KS1.iam
- C:\Users\Cosmonauta\ownCloud\Aurora\Proyectos\SUCHAI_2-3\Subsistemas\MEC\CAD_Cubesat3U\Nanopower_P31U\CAD\KS2.iam
- C:\Users\Cosmonauta\ownCloud\Aurora\Proyectos\SUCHAI_2-3\Subsistemas\MEC\CAD_Cubesat3U\Nanopower_P31U\CAD\R607.iam
- C:\Users\Cosmonauta\ownCloud\Aurora\Proyectos\SUCHAI_2-3\Subsistemas\MEC\CAD_Cubesat3U\Nanopower_P31U\CAD\R608.iam
- C:\Users\Cosmonauta\ownCloud\Aurora\Proyectos\SUCHAI_2-3\Subsistemas\MEC\CAD_Cubesat3U\Nanopower_P31U\CAD\R609.iam
- C:\Users\Cosmonauta\ownCloud\Aurora\Proyectos\SUCHAI_2-3\Subsistemas\MEC\CAD_Cubesat3U\Nanopower_P31U\CAD\R610.iam
- C:\Users\Cosmonauta\ownCloud\Aurora\Proyectos\SUCHAI_2-3\Subsistemas\MEC\CAD_Cubesat3U\Nanopower_P31U\CAD\R611.iam
- C:\Users\Cosmonauta\ownCloud\Aurora\Proyectos\SUCHAI_2-3\Subsistemas\MEC\CAD_Cubesat3U\Nanopower_P31U\CAD\R612.iam
- C:\Users\Cosmonauta\ownCloud\Aurora\Proyectos\SUCHAI_2-3\Subsistemas\MEC\CAD_Cubesat3U\Nanopower_P31U\CAD\R613.iam
- C:\Users\Cosmonauta\ownCloud\Aurora\Proyectos\SUCHAI_2-3\Subsistemas\MEC\CAD_Cubesat3U\Nanopower_P31U\CAD\R614.iam
- C:\Users\Cosmonauta\ownCloud\Aurora\Proyectos\SUCHAI_2-3\Subsistemas\MEC\CAD_Cubesat3U\Nanopower_P31U\CAD\R615.iam
- C:\Users\Cosmonauta\ownCloud\Aurora\Proyectos\SUCHAI_2-3\Subsistemas\MEC\CAD_Cubesat3U\Nanopower_P31U\CAD\R616.iam
- C:\Users\Cosmonauta\ownCloud\Aurora\Proyectos\SUCHAI_2-3\Subsistemas\MEC\CAD_Cubesat3U\Nanopower_P31U\CAD\R617.iam
- C:\Users\Cosmonauta\ownCloud\Aurora\Proyectos\SUCHAI_2-3\Subsistemas\MEC\CAD_Cubesat3U\Nanopower_P31U\CAD\R618.iam
- C:\Users\Cosmonauta\ownCloud\Aurora\Proyectos\SUCHAI_2-3\Subsistemas\MEC\CAD_Cubesat3U\Nanopower_P31U\CAD\U203.iam
- C:\Users\Cosmonauta\ownCloud\Aurora\Proyectos\SUCHAI_2-3\Subsistemas\MEC\CAD_Cubesat3U\Nanopower_P31U\CAD\R301.iam
- C:\Users\Cosmonauta\ownCloud\Aurora\Proyectos\SUCHAI_2-3\Subsistemas\MEC\CAD_Cubesat3U\Nanopower_P31U\CAD\R302.iam
- C:\Users\Cosmonauta\ownCloud\Aurora\Proyectos\SUCHAI_2-3\Subsistemas\MEC\CAD_Cubesat3U\Nanopower_P31U\CAD\PBAT1.iam
- C:\Users\Cosmonauta\ownCloud\Aurora\Proyectos\SUCHAI_2-3\Subsistemas\MEC\CAD_Cubesat3U\Nanopower_P31U\CAD\U606.iam
- C:\Users\Cosmonauta\ownCloud\Aurora\Proyectos\SUCHAI_2-3\Subsistemas\MEC\CAD_Cubesat3U\Nanopower_P31U\CAD\U607.iam
- C:\Users\Cosmonauta\ownCloud\Aurora\Proyectos\SUCHAI_2-3\Subsistemas\MEC\CAD_Cubesat3U\Nanopower_P31U\CAD\R624.iam
- C:\Users\Cosmonauta\ownCloud\Aurora\Proyectos\SUCHAI_2-3\Subsistemas\MEC\CAD_Cubesat3U\Nanopower_P31U\CAD\R625.iam
- C:\Users\Cosmonauta\ownCloud\Aurora\Proyectos\SUCHAI_2-3\Subsistemas\MEC\CAD_Cubesat3U\Nanopower_P31U\CAD\P107.iam
- C:\Users\Cosmonauta\ownCloud\Aurora\Proyectos\SUCHAI_2-3\Subsistemas\MEC\CAD_Cubesat3U\Nanopower_P31U\CAD\R415.iam
- C:\Users\Cosmonauta\ownCloud\Aurora\Proyectos\SUCHAI_2-3\Subsistemas\MEC\CAD_Cubesat3U\Nanopower_P31U\CAD\R416.iam
- C:\Users\Cosmonauta\ownCloud\Aurora\Proyectos\SUCHAI_2-3\Subsistemas\MEC\CAD_Cubesat3U\Nanopower_P31U\CAD\R417.iam
- C:\Users\Cosmonauta\ownCloud\Aurora\Proyectos\SUCHAI_2-3\Subsistemas\MEC\CAD_Cubesat3U\Nanopower_P31U\CAD\U400.iam
- C:\Users\Cosmonauta\ownCloud\Aurora\Proyectos\SUCHAI_2-3\Subsistemas\MEC\CAD_Cubesat3U\Nanopower_P31U\CAD\R211.iam
- C:\Users\Cosmonauta\ownCloud\Aurora\Proyectos\SUCHAI_2-3\Subsistemas\MEC\CAD_Cubesat3U\Nanopower_P31U\CAD\R212.iam
- C:\Users\Cosmonauta\ownCloud\Aurora\Proyectos\SUCHAI_2-3\Subsistemas\MEC\CAD_Cubesat3U\Nanopower_P31U\CAD\U202.iam
- C:\Users\Cosmonauta\ownCloud\Aurora\Proyectos\SUCHAI_2-3\Subsistemas\MEC\CAD_Cubesat3U\Nanopower_P31U\CAD\BT1.iam
- C:\Users\Cosmonauta\ownCloud\Aurora\Proyectos\SUCHAI_2-3\Subsistemas\MEC\CAD_Cubesat3U\Nanopower_P31U\CAD\C67.iam
- C:\Users\Cosmonauta\ownCloud\Aurora\Proyectos\SUCHAI_2-3\Subsistemas\MEC\CAD_Cubesat3U\Nanopower_P31U\CAD\R27.iam
- C:\Users\Cosmonauta\ownCloud\Aurora\Proyectos\SUCHAI_2-3\Subsistemas\MEC\CAD_Cubesat3U\Nanopower_P31U\CAD\R29.iam
- C:\Users\Cosmonauta\ownCloud\Aurora\Proyectos\SUCHAI_2-3\Subsistemas\MEC\CAD_Cubesat3U\Nanopower_P31U\CAD\R30.iam